# Autodesk Inventor assembly: nozzle
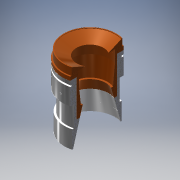
[picture p0: Inventor's stored thumbnail of the model, 180x180]
Saved by Autodesk Inventor 2017 SP1 (Build 210196100, 196)
## iProperties
Created: 2016-10-29
Part Number: nozzle
Document SubType Name: Assembly
Designer: cflannery
Author: cflannery
## Documents named in this file (6)
- D:\Triton_Rocket_Club\Propulsion\Launches\8-inch-flight\Design\CAD\Vehicle\Nozzle\trunk\nozzle.iam
- D:\Triton_Rocket_Club\Propulsion\Launches\8-inch-flight\Design\CAD\Vehicle\Nozzle\trunk\aluminum_casing.ipt
- D:\Triton_Rocket_Club\Propulsion\Launches\8-inch-flight\Design\CAD\Vehicle\Nozzle\trunk\aluminum_retainer.ipt
- D:\Triton_Rocket_Club\Propulsion\Launches\8-inch-flight\Design\CAD\Vehicle\Nozzle\trunk\aluminum_skirt.ipt
- D:\Triton_Rocket_Club\Propulsion\Launches\8-inch-flight\Design\CAD\Vehicle\Nozzle\trunk\phenolic_bottom.ipt
- D:\Triton_Rocket_Club\Propulsion\Launches\8-inch-flight\Design\CAD\Vehicle\Nozzle\trunk\phenolic_top.ipt
## Components (5 placed, 5 different names)
1. aluminum_casing:1 — Mate:8, Mate:9, Mate:10, Mate:14, Mate:15
2. aluminum_retainer:1 — Mate:9, Mate:14
3. aluminum_skirt:1 — Mate:10, Mate:15
4. phenolic_bottom:1 — Mate:7
5. phenolic_top:1 — Mate:7, Mate:8
## Relationships (6: Mate 6)
- Mate:7: phenolic_bottom:1 ↔ phenolic_top:1
- Mate:8: aluminum_casing:1 ↔ phenolic_top:1
- Mate:9: aluminum_casing:1 ↔ aluminum_retainer:1
- Mate:10: aluminum_casing:1 ↔ aluminum_skirt:1
- Mate:14: aluminum_casing:1 ↔ aluminum_retainer:1
- Mate:15: aluminum_casing:1 ↔ aluminum_skirt:1
